# Autodesk Inventor assembly: ПД Модуль 200х140х75
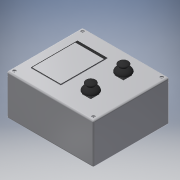
[picture p0: Inventor's stored thumbnail of the model, 180x180]
Saved by Autodesk Inventor 2019 (Build 230136000, 136)
## iProperties
Created: 2020-05-19
Part Number: ПД Модуль 200х140х75
Material: Типовые
Document SubType Name: Assembly
Designer: Surflay
Author: Surflay
## Documents named in this file (10)
- C:\Users\Surflay\Desktop\Документы\Университет\5 семестр\ПД\Модуль ДУ Inventor\Дистанционная связь (модуль)\ПД Модуль 200х140х75.iam
- C:\Users\Surflay\Desktop\Документы\Университет\5 семестр\ПД\Модуль ДУ Inventor\Дистанционная связь (модуль)\ПД Коробка 160х140х75.ipt
- C:\Users\Surflay\Desktop\Документы\Университет\5 семестр\ПД\Модуль ДУ Inventor\Дистанционная связь (модуль)\Каркас.ipt
- C:\Users\Surflay\Desktop\Документы\Университет\5 семестр\ПД\Модуль ДУ Inventor\Дистанционная связь (модуль)\РадиоМодуль.ipt
- C:\Users\Surflay\Desktop\Документы\Университет\5 семестр\ПД\Модуль ДУ Inventor\Дистанционная связь (модуль)\Arduino UNO.ipt
- C:\Users\Surflay\Desktop\Документы\Университет\5 семестр\ПД\Модуль ДУ Inventor\Дистанционная связь (модуль)\Аккумулятор.ipt
- C:\Users\Surflay\Desktop\Документы\Университет\5 семестр\ПД\Модуль ДУ Inventor\Дистанционная связь (модуль)\Кнопка.ipt
- C:\Users\Surflay\Desktop\Документы\Университет\5 семестр\ПД\Модуль ДУ Inventor\Дистанционная связь (модуль)\ВольтметрЦифровой.ipt
- C:\Users\Surflay\Desktop\Документы\Университет\5 семестр\ПД\Модуль ДУ Inventor\Дистанционная связь (модуль)\NextionDisplay.ipt
- C:\Users\Surflay\Desktop\Документы\Университет\5 семестр\ПД\Модуль ДУ Inventor\Дистанционная связь (модуль)\Джойстик.ipt
## Components (10 placed, 9 different names)
1. ПД Коробка 160х140х75:1 — Совмещение:6, Совмещение:10, Совмещение:11, Совмещение:14, Совмещение:16, Совмещение:17, Совмещение:19, Совмещение:20, Совмещение:22, Совмещение:23, Совмещение:26, Совмещение:27, Совмещение:28, Совмещение:29, Совмещение:30, Совмещение:31
2. Каркас:1 — Совмещение:6, Угол:8, Совмещение:12, Совмещение:13, Совмещение:15, Совмещение:21, Совмещение:24, Совмещение:25
3. РадиоМодуль:1 — Угол:8, Совмещение:10, Совмещение:11, Совмещение:12
4. Arduino UNO:1 — Совмещение:13, Совмещение:14, Совмещение:15
5. Аккумулятор:1 — Совмещение:16, Совмещение:17, Совмещение:25
6. Кнопка:1 — Совмещение:19, Совмещение:20, Совмещение:21
7. ВольтметрЦифровой:1 — Совмещение:22, Совмещение:23, Совмещение:24
8. NextionDisplay:1 — Совмещение:26, Совмещение:27, Совмещение:28
9. Джойстик:1 — Совмещение:29, Совмещение:30, Совмещение:31
10. Джойстик:2
## Component patterns: (2 elements, first: Джойстик:1)
## Relationships (23: Mate 22, Angle 1)
- Совмещение:6 [Mate]: ПД Коробка 160х140х75:1 ↔ Каркас:1
- Угол:8 [Angle] (180 deg): Каркас:1 ↔ РадиоМодуль:1
- Совмещение:10 [Mate] (30 mm): ПД Коробка 160х140х75:1 ↔ РадиоМодуль:1
- Совмещение:11 [Mate] (109 mm): ПД Коробка 160х140х75:1 ↔ РадиоМодуль:1
- Совмещение:12 [Mate]: Каркас:1 ↔ РадиоМодуль:1
- Совмещение:13 [Mate]: Каркас:1 ↔ Arduino UNO:1
- Совмещение:14 [Mate]: ПД Коробка 160х140х75:1 ↔ Arduino UNO:1
- Совмещение:15 [Mate]: Каркас:1 ↔ Arduino UNO:1
- Совмещение:16 [Mate] (12 mm): ПД Коробка 160х140х75:1 ↔ Аккумулятор:1
- Совмещение:17 [Mate] (8 mm): ПД Коробка 160х140х75:1 ↔ Аккумулятор:1
- Совмещение:19 [Mate]: ПД Коробка 160х140х75:1 ↔ Кнопка:1
- Совмещение:20 [Mate] (25 mm): ПД Коробка 160х140х75:1 ↔ Кнопка:1
- Совмещение:21 [Mate] (15 mm): Каркас:1 ↔ Кнопка:1
- Совмещение:22 [Mate]: ПД Коробка 160х140х75:1 ↔ ВольтметрЦифровой:1
- Совмещение:23 [Mate] (57 mm): ПД Коробка 160х140х75:1 ↔ ВольтметрЦифровой:1
- Совмещение:24 [Mate] (9 mm): Каркас:1 ↔ ВольтметрЦифровой:1
- Совмещение:25 [Mate]: Каркас:1 ↔ Аккумулятор:1
- Совмещение:26 [Mate]: ПД Коробка 160х140х75:1 ↔ NextionDisplay:1
- Совмещение:27 [Mate] (15 mm): ПД Коробка 160х140х75:1 ↔ NextionDisplay:1
- Совмещение:28 [Mate] (15 mm): ПД Коробка 160х140х75:1 ↔ NextionDisplay:1
- Совмещение:29 [Mate] (5 mm): ПД Коробка 160х140х75:1 ↔ Джойстик:1
- Совмещение:30 [Mate] (25 mm): ПД Коробка 160х140х75:1 ↔ Джойстик:1
- Совмещение:31 [Mate] (30 mm): ПД Коробка 160х140х75:1 ↔ Джойстик:1
